# Autodesk Inventor assembly: Zebro_z_lotka
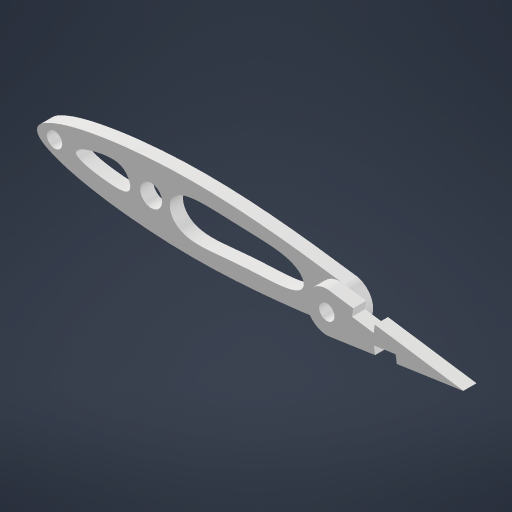
[picture p0: Inventor's stored thumbnail of the model, 512x512]
Saved by Autodesk Inventor 2023 (Build 270158000, 158)
## iProperties
Created: 2023-01-05
Part Number: Zebro_z_lotka
Document SubType Name: Assembly
Designer: szykr
Author: szykr
## Documents named in this file (3)
- D:\Folder Instalacyjny\GitHub Pliki\Solaris\new model\Tail\Zebro_z_lotka.iam
- D:\Folder Instalacyjny\GitHub Pliki\Solaris\new model\Tail\Tżebro z lotkąt.ipt
- D:\Folder Instalacyjny\GitHub Pliki\Solaris\new model\Tail\Tlotka.ipt
## Components (2 placed, 2 different names)
1. Tżebro z lotkąt:1 — Insert:1
2. Tlotka:1 — Insert:1
## Relationships (1: Insert 1)
- Insert:1: Tżebro z lotkąt:1 ↔ Tlotka:1
